# Autodesk Inventor assembly: Pickle Floorplan
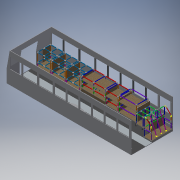
[picture p0: Inventor's stored thumbnail of the model, 180x180]
Saved by Autodesk Inventor 2018.2 (Build 222227000, 227)
## iProperties
Created: 2018-02-27
Part Number: Pickle Floorplan
Document SubType Name: Assembly
Designer: owner
Author: owner
## Documents named in this file (17)
- Z:\The Pickle\Final Carts\Pickle Floorplan.iam
- Z:\The Pickle\Final Carts\Pickle Interior Assembly\Pickle Interior.ipt
- Z:\The Pickle\Final Carts\Mellie Cart\Mellie Cart.iam
- Z:\The Pickle\Final Carts\T-Bone Cart\TBone Cart.iam
- Z:\The Pickle\Final Carts\Sax Cart\Bari Cart.iam
- Z:\The Pickle\Final Carts\Sax Cart\Tenor Cart OPTION 2.iam
- Z:\The Pickle\Final Carts\Euph Cart\Euph Cart.iam
- Z:\The Pickle\Final Carts\Mellie Cart\Mellie Side Cart.iam
- Z:\The Pickle\Final Carts\Sax Cart\Tenor Sax Mounting eyenut.ipt
- Z:\The Pickle\Final Carts\Sax Cart\Tenor Sax Mounting Screw.ipt
- Z:\The Pickle\Final Carts\Locking Mech\euph tenor mount\euph tenor plywood mount.iam
- Z:\The Pickle\Final Carts\Locking Mech\mellie side cart mounts\mellie side count plywood mounts.iam
- Z:\The Pickle\Final Carts\Locking Mech\t-bone and mellie mount\t-bone and mellie plywood mount.iam
- Z:\The Pickle\Final Carts\Locking Mech\t-bone mount\T-bone plywood mount.iam
- Z:\The Pickle\Final Carts\Locking Mech\tenor mount\tenor plywood mount.iam
- Z:\The Pickle\Final Carts\Locking Mech\Eyebolt for wood.ipt
- Z:\The Pickle\Final Carts\Locking Mech\t-bone end mount\t-bone end plywood mount.iam
## Components (50 placed, 16 different names)
1. Pickle Interior:1 — Mate:2, Mate:3, Mate:4, Mate:7, Mate:8, Tangent:1, Mate:10, Tangent:3, Tangent:4, Tangent:5, Mate:13, Mate:14, Mate:15, Tangent:6, Tangent:7, Tangent:8, Tangent:9, Tangent:10, Tangent:11, Mate:69, Mate:70, Mate:75, Mate:78, Mate:79
2. euph tenor plywood mount:1 [sub-assembly] — Flush:3, Flush:4, Flush:15, Flush:16
3. mellie side count plywood mounts:1 [sub-assembly] — Flush:4, Flush:5, Flush:14, Flush:15
4. mellie side count plywood mounts:2 [sub-assembly] — Flush:5, Flush:6, Flush:13, Flush:14
5. t-bone and mellie plywood mount:1 [sub-assembly] — Flush:6, Flush:7, Flush:12, Flush:13
6. T-bone plywood mount:1 [sub-assembly] — Flush:7, Flush:8, Flush:11, Flush:12
7. T-bone plywood mount:2 [sub-assembly] — Flush:8, Flush:11
8. tenor plywood mount:1 [sub-assembly] — Flush:3, Flush:16, Mate:69, Mate:70
9. Eyebolt for wood:2 — Angle:8, Mate:73, Mate:75
10. t-bone end plywood mount:1 [sub-assembly] — Mate:78, Mate:79
11. Mellie Cart:1 [sub-assembly] — Mate:10, Mate:13, Angle:4, Tangent:27, Mate:34, Tangent:28, Tangent:29, Mate:37, Tangent:30, Tangent:31
12. TBone Cart:1 [sub-assembly] — Mate:4, Flush:1, Tangent:4, Tangent:5, Mate:16, Mate:17, Tangent:12, Tangent:13, Mate:19, Angle:1, Tangent:14, Tangent:15, Tangent:16
13. TBone Cart:2 [sub-assembly] — Mate:3, Flush:2, Angle:3, Tangent:22, Mate:28, Tangent:23, Tangent:24, Angle:9, Tangent:51, Mate:77, Tangent:52, Tangent:53
14. TBone Cart:3 [sub-assembly] — Mate:2, Flush:1, Flush:2, Mate:22, Angle:2, Tangent:17, Tangent:18, Tangent:19, Mate:25, Tangent:20, Tangent:21
15. Bari Cart:1 [sub-assembly] — Mate:7, Tangent:1, Tangent:3, Mate:58, Tangent:46, Tangent:47, Angle:7, Tangent:48, Tangent:49, Tangent:50
16. Tenor Cart OPTION 2:1 [sub-assembly] — Mate:8, Tangent:10, Tangent:11, Mate:52, Mate:53, Tangent:42, Tangent:43, Mate:55, Tangent:44, Mate:56, Tangent:45
17. Euph Cart:1 [sub-assembly] — Mate:14, Tangent:8, Tangent:9, Angle:6, Tangent:37, Mate:46, Tangent:38, Tangent:39, Mate:49, Tangent:40, Tangent:41
18. Mellie Side Cart:1 [sub-assembly] — Mate:15, Tangent:6, Tangent:7, Angle:5, Tangent:32, Mate:40, Tangent:33, Tangent:34, Mate:43, Tangent:35, Tangent:36
19. Tenor Sax Mounting eyenut:1 — Mate:33, Tangent:53
20. Tenor Sax Mounting Screw:1 — Mate:33, Mate:76, Mate:77, Tangent:52
21. Tenor Sax Mounting eyenut:2 — Tangent:16, Mate:21
22. Tenor Sax Mounting Screw:2 — Mate:19, Mate:20, Tangent:15, Mate:21
23. Tenor Sax Mounting eyenut:3 — Mate:27, Tangent:21
24. Tenor Sax Mounting Screw:3 — Mate:25, Mate:26, Tangent:20, Mate:27
25. Tenor Sax Mounting eyenut:4 — Tangent:19, Mate:24
26. Tenor Sax Mounting Screw:4 — Mate:16, Mate:17, Tangent:12, Mate:18
27. Tenor Sax Mounting eyenut:5 — Tangent:13, Mate:18
28. Tenor Sax Mounting Screw:5 — Mate:22, Mate:23, Tangent:18, Mate:24
29. Tenor Sax Mounting eyenut:6 — Tangent:24, Mate:30
30. Tenor Sax Mounting Screw:6 — Mate:28, Mate:29, Tangent:23, Mate:30
31. Tenor Sax Mounting Screw:11 — Mate:58, Tangent:46, Mate:60, Mate:61, Mate:62, Mate:74
32. Tenor Sax Mounting Screw:12 — Mate:55, Tangent:44, Mate:56, Mate:57
33. Tenor Sax Mounting Screw:13 — Mate:49, Mate:50, Tangent:40, Mate:51
34. Tenor Sax Mounting Screw:14 — Mate:43, Mate:44, Tangent:35, Mate:45
35. Tenor Sax Mounting Screw:15 — Mate:37, Mate:38, Tangent:30, Mate:39
36. Tenor Sax Mounting Screw:16 — Mate:62, Tangent:49, Mate:63
37. Tenor Sax Mounting Screw:20 — Mate:52, Mate:53, Tangent:42, Mate:54
38. Tenor Sax Mounting Screw:21 — Mate:46, Mate:47, Tangent:38, Mate:48
39. Tenor Sax Mounting Screw:22 — Mate:40, Mate:41, Tangent:33, Mate:42
40. Tenor Sax Mounting Screw:23 — Mate:34, Mate:35, Tangent:28, Mate:36
41. Tenor Sax Mounting eyenut:10 — Mate:60, Tangent:47
42. Tenor Sax Mounting eyenut:11 — Mate:57, Tangent:45
43. Tenor Sax Mounting eyenut:12 — Mate:51, Tangent:41
44. Tenor Sax Mounting eyenut:13 — Mate:45, Tangent:36
45. Tenor Sax Mounting eyenut:14 — Mate:39, Tangent:31
46. Tenor Sax Mounting eyenut:15 — Mate:36, Tangent:29
47. Tenor Sax Mounting eyenut:16 — Mate:42, Tangent:34
48. Tenor Sax Mounting eyenut:17 — Mate:48, Tangent:39
49. Tenor Sax Mounting eyenut:18 — Mate:54, Tangent:43
50. Tenor Sax Mounting eyenut:22 — Tangent:50, Mate:63
## Relationships (136: Mate 63, Tangent 50, Flush 14, Angle 9)
- Mate:2 (120.65 mm): Pickle Interior:1 ↔ TBone Cart:3
- Mate:3 (120.65 mm): Pickle Interior:1 ↔ TBone Cart:2
- Mate:4 (120.65 mm): Pickle Interior:1 ↔ TBone Cart:1
- Mate:7 (73.025 mm): Pickle Interior:1 ↔ Bari Cart:1
- Mate:8 (120.65 mm): Pickle Interior:1 ↔ Tenor Cart OPTION 2:1
- Tangent:1: Pickle Interior:1 ↔ Bari Cart:1
- Flush:1: TBone Cart:1 ↔ TBone Cart:3
- Flush:2: TBone Cart:2 ↔ TBone Cart:3
- Mate:10: Pickle Interior:1 ↔ Mellie Cart:1
- Tangent:3: Pickle Interior:1 ↔ Bari Cart:1
- Tangent:4: Pickle Interior:1 ↔ TBone Cart:1
- Tangent:5: Pickle Interior:1 ↔ TBone Cart:1
- Mate:13 (247.65 mm): Pickle Interior:1 ↔ Mellie Cart:1
- Mate:14 (120.65 mm): Pickle Interior:1 ↔ Euph Cart:1
- Mate:15 (120.65 mm): Pickle Interior:1 ↔ Mellie Side Cart:1
- Tangent:6 (17.907 mm): Pickle Interior:1 ↔ Mellie Side Cart:1
- Tangent:7 (17.907 mm): Pickle Interior:1 ↔ Mellie Side Cart:1
- Tangent:8 (17.907 mm): Pickle Interior:1 ↔ Euph Cart:1
- Tangent:9 (17.907 mm): Pickle Interior:1 ↔ Euph Cart:1
- Tangent:10 (5.0546 mm): Pickle Interior:1 ↔ Tenor Cart OPTION 2:1
- Tangent:11 (5.0546 mm): Pickle Interior:1 ↔ Tenor Cart OPTION 2:1
- Mate:16 (20.1676 mm): TBone Cart:1 ↔ Tenor Sax Mounting Screw:4
- Mate:17 (-16.7132 mm): TBone Cart:1 ↔ Tenor Sax Mounting Screw:4
- Tangent:12: TBone Cart:1 ↔ Tenor Sax Mounting Screw:4
- Tangent:13: TBone Cart:1 ↔ Tenor Sax Mounting eyenut:5
- Mate:18: Tenor Sax Mounting Screw:4 ↔ Tenor Sax Mounting eyenut:5
- Mate:19 (12.7 mm): TBone Cart:1 ↔ Tenor Sax Mounting Screw:2
- Angle:1 (0 deg): TBone Cart:1
- Tangent:14: TBone Cart:1
- Mate:20 (-16.7132 mm): Tenor Sax Mounting Screw:2
- Tangent:15: TBone Cart:1 ↔ Tenor Sax Mounting Screw:2
- Tangent:16: TBone Cart:1 ↔ Tenor Sax Mounting eyenut:2
- Mate:21: Tenor Sax Mounting eyenut:2 ↔ Tenor Sax Mounting Screw:2
- Mate:22 (38.1 mm): TBone Cart:3 ↔ Tenor Sax Mounting Screw:5
- Angle:2 (0 deg): TBone Cart:3
- Tangent:17: TBone Cart:3
- Mate:23 (-16.7132 mm): Tenor Sax Mounting Screw:5
- Tangent:18: TBone Cart:3 ↔ Tenor Sax Mounting Screw:5
- Tangent:19: TBone Cart:3 ↔ Tenor Sax Mounting eyenut:4
- Mate:24: Tenor Sax Mounting eyenut:4 ↔ Tenor Sax Mounting Screw:5
- Mate:25 (12.7 mm): TBone Cart:3 ↔ Tenor Sax Mounting Screw:3
- Mate:26 (-16.7132 mm): Tenor Sax Mounting Screw:3
- Tangent:20: TBone Cart:3 ↔ Tenor Sax Mounting Screw:3
- Mate:27: Tenor Sax Mounting eyenut:3 ↔ Tenor Sax Mounting Screw:3
- Tangent:21: TBone Cart:3 ↔ Tenor Sax Mounting eyenut:3
- Angle:3 (0 deg): TBone Cart:2
- Tangent:22: TBone Cart:2
- Mate:28 (38.1 mm): TBone Cart:2 ↔ Tenor Sax Mounting Screw:6
- Mate:29 (-16.7132 mm): Tenor Sax Mounting Screw:6
- Tangent:23: TBone Cart:2 ↔ Tenor Sax Mounting Screw:6
- Tangent:24: TBone Cart:2 ↔ Tenor Sax Mounting eyenut:6
- Mate:30: Tenor Sax Mounting eyenut:6 ↔ Tenor Sax Mounting Screw:6
- Mate:33: Tenor Sax Mounting eyenut:1 ↔ Tenor Sax Mounting Screw:1
- Angle:4 (0 deg): Mellie Cart:1
- Tangent:27: Mellie Cart:1
- Mate:34 (25.4 mm): Mellie Cart:1 ↔ Tenor Sax Mounting Screw:23
- Mate:35 (16.7132 mm): Tenor Sax Mounting Screw:23
- Tangent:28: Mellie Cart:1 ↔ Tenor Sax Mounting Screw:23
- Mate:36: Tenor Sax Mounting Screw:23 ↔ Tenor Sax Mounting eyenut:15
- Tangent:29: Mellie Cart:1 ↔ Tenor Sax Mounting eyenut:15
- Mate:37 (25.4 mm): Mellie Cart:1 ↔ Tenor Sax Mounting Screw:15
- Mate:38 (16.7132 mm): Tenor Sax Mounting Screw:15
- Tangent:30: Mellie Cart:1 ↔ Tenor Sax Mounting Screw:15
- Mate:39: Tenor Sax Mounting Screw:15 ↔ Tenor Sax Mounting eyenut:14
- Tangent:31: Mellie Cart:1 ↔ Tenor Sax Mounting eyenut:14
- Angle:5 (0 deg): Mellie Side Cart:1
- Tangent:32: Mellie Side Cart:1
- Mate:40 (25.4 mm): Mellie Side Cart:1 ↔ Tenor Sax Mounting Screw:22
- Mate:41 (16.7132 mm): Tenor Sax Mounting Screw:22
- Tangent:33: Mellie Side Cart:1 ↔ Tenor Sax Mounting Screw:22
- Mate:42: Tenor Sax Mounting Screw:22 ↔ Tenor Sax Mounting eyenut:16
- Tangent:34: Mellie Side Cart:1 ↔ Tenor Sax Mounting eyenut:16
- Mate:43 (25.4 mm): Mellie Side Cart:1 ↔ Tenor Sax Mounting Screw:14
- Mate:44 (16.7132 mm): Tenor Sax Mounting Screw:14
- Tangent:35: Mellie Side Cart:1 ↔ Tenor Sax Mounting Screw:14
- Mate:45: Tenor Sax Mounting Screw:14 ↔ Tenor Sax Mounting eyenut:13
- Tangent:36: Mellie Side Cart:1 ↔ Tenor Sax Mounting eyenut:13
- Angle:6 (0 deg): Euph Cart:1
- Tangent:37: Euph Cart:1
- Mate:46 (127 mm): Euph Cart:1 ↔ Tenor Sax Mounting Screw:21
- Mate:47 (16.7132 mm): Tenor Sax Mounting Screw:21
- Tangent:38: Euph Cart:1 ↔ Tenor Sax Mounting Screw:21
- Mate:48: Tenor Sax Mounting Screw:21 ↔ Tenor Sax Mounting eyenut:17
- Tangent:39: Euph Cart:1 ↔ Tenor Sax Mounting eyenut:17
- Mate:49 (76.2 mm): Euph Cart:1 ↔ Tenor Sax Mounting Screw:13
- Mate:50 (16.7132 mm): Tenor Sax Mounting Screw:13
- Tangent:40: Euph Cart:1 ↔ Tenor Sax Mounting Screw:13
- Mate:51: Tenor Sax Mounting Screw:13 ↔ Tenor Sax Mounting eyenut:12
- Tangent:41: Euph Cart:1 ↔ Tenor Sax Mounting eyenut:12
- Mate:52 (12.5476 mm): Tenor Cart OPTION 2:1 ↔ Tenor Sax Mounting Screw:20
- Mate:53 (-16.7132 mm): Tenor Cart OPTION 2:1 ↔ Tenor Sax Mounting Screw:20
- Tangent:42: Tenor Cart OPTION 2:1 ↔ Tenor Sax Mounting Screw:20
- Mate:54: Tenor Sax Mounting Screw:20 ↔ Tenor Sax Mounting eyenut:18
- Tangent:43: Tenor Cart OPTION 2:1 ↔ Tenor Sax Mounting eyenut:18
- Mate:55 (12.7 mm): Tenor Cart OPTION 2:1 ↔ Tenor Sax Mounting Screw:12
- Tangent:44: Tenor Cart OPTION 2:1 ↔ Tenor Sax Mounting Screw:12
- Mate:56 (-16.7132 mm): Tenor Cart OPTION 2:1 ↔ Tenor Sax Mounting Screw:12
- Mate:57: Tenor Sax Mounting Screw:12 ↔ Tenor Sax Mounting eyenut:11
- Tangent:45: Tenor Cart OPTION 2:1 ↔ Tenor Sax Mounting eyenut:11
- Mate:58 (25.4 mm): Bari Cart:1 ↔ Tenor Sax Mounting Screw:11
- Tangent:46: Bari Cart:1 ↔ Tenor Sax Mounting Screw:11
- Mate:60: Tenor Sax Mounting Screw:11 ↔ Tenor Sax Mounting eyenut:10
- Tangent:47: Bari Cart:1 ↔ Tenor Sax Mounting eyenut:10
- Angle:7 (0 deg): Bari Cart:1
- Tangent:48: Bari Cart:1
- Mate:61 (16.7132 mm): Tenor Sax Mounting Screw:11
- Mate:62: Tenor Sax Mounting Screw:11 ↔ Tenor Sax Mounting Screw:16
- Tangent:49: Bari Cart:1 ↔ Tenor Sax Mounting Screw:16
- Tangent:50: Bari Cart:1 ↔ Tenor Sax Mounting eyenut:22
- Mate:63: Tenor Sax Mounting Screw:16 ↔ Tenor Sax Mounting eyenut:22
- Flush:3: euph tenor plywood mount:1 ↔ tenor plywood mount:1
- Flush:4: euph tenor plywood mount:1 ↔ mellie side count plywood mounts:1
- Flush:5: mellie side count plywood mounts:1 ↔ mellie side count plywood mounts:2
- Flush:6: mellie side count plywood mounts:2 ↔ t-bone and mellie plywood mount:1
- Flush:7: t-bone and mellie plywood mount:1 ↔ T-bone plywood mount:1
- Flush:8: T-bone plywood mount:1 ↔ T-bone plywood mount:2
- Flush:11: T-bone plywood mount:1 ↔ T-bone plywood mount:2
- Flush:12: t-bone and mellie plywood mount:1 ↔ T-bone plywood mount:1
- Flush:13: mellie side count plywood mounts:2 ↔ t-bone and mellie plywood mount:1
- Flush:14: mellie side count plywood mounts:1 ↔ mellie side count plywood mounts:2
- Flush:15: euph tenor plywood mount:1 ↔ mellie side count plywood mounts:1
- Flush:16: euph tenor plywood mount:1 ↔ tenor plywood mount:1
- Mate:69: Pickle Interior:1 ↔ tenor plywood mount:1
- Mate:70: Pickle Interior:1 ↔ tenor plywood mount:1
- Angle:8 (0 deg): Eyebolt for wood:2
- Mate:73: Eyebolt for wood:2
- Mate:74: Tenor Sax Mounting Screw:11
- Mate:75: Pickle Interior:1 ↔ Eyebolt for wood:2
- Angle:9 (0 deg): TBone Cart:2
- Tangent:51: TBone Cart:2
- Mate:76 (-16.7132 mm): Tenor Sax Mounting Screw:1
- Mate:77 (25.4 mm): TBone Cart:2 ↔ Tenor Sax Mounting Screw:1
- Tangent:52: TBone Cart:2 ↔ Tenor Sax Mounting Screw:1
- Tangent:53: TBone Cart:2 ↔ Tenor Sax Mounting eyenut:1
- Mate:78: Pickle Interior:1 ↔ t-bone end plywood mount:1
- Mate:79: Pickle Interior:1 ↔ t-bone end plywood mount:1
